# Autodesk Inventor assembly: LifterRight
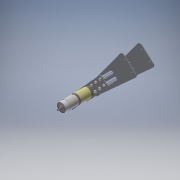
[picture p0: Inventor's stored thumbnail of the model, 180x180]
Saved by Autodesk Inventor 2017 (Build 210142000, 142)
## iProperties
Created: 2017-02-09
Part Number: LifterRight
Document SubType Name: Assembly
Designer: kingb
Author: kingb
## Documents named in this file (10)
- C:\Users\kingb\Desktop\CAD\LifterRight.iam
- C:\Users\kingb\Desktop\CAD\lifterMountMetal.ipt
- C:\Users\kingb\Desktop\CAD\newCoupler.ipt
- C:\Users\kingb\Desktop\CAD\Churro 3375.ipt
- C:\Users\kingb\Desktop\CAD\guidebar.ipt
- C:\Users\kingb\Desktop\CAD\10-32x0500_shcs_HX-SHCS 0.19-32x1.375x1-C.ipt
- C:\Users\kingb\Desktop\CAD\FHTS 0.25-20-0.75_FHTS 0.25-20-G-0.75-C.ipt
- C:\Users\kingb\Desktop\CAD\10-32 Nylock Nut.ipt
- C:\Users\kingb\Desktop\CAD\PG188withMotor.ipt
- C:\Users\kingb\Desktop\CAD\pG188Mount.ipt
## Components (30 placed, 9 different names)
1. lifterMountMetal:1 — Mate:5, Mate:6, Insert:12, Insert:14, Insert:15, Insert:16, Insert:17, Insert:26, Insert:27, Mate:11, Mate:12, Insert:30, Mate:18
2. newCoupler:1
3. Churro 3375:1 — Insert:31
4. Churro 3375:2 — Insert:34
5. Churro 3375:3 — Mate:5, Insert:33
6. Churro 3375:5 — Insert:32
7. guidebar:1 — Mate:6, Insert:24, Insert:25, Insert:28, Insert:29, Mate:11, Mate:12
8. Churro 3375:6 — Insert:36
9. Churro 3375:7 — Insert:35
10. 10-32x0500_shcs_HX-SHCS 0.19-32x1.375x1-C:1
11. 10-32x0500_shcs_HX-SHCS 0.19-32x1.375x1-C:2
12. FHTS 0.25-20-0.75_FHTS 0.25-20-G-0.75-C:1
13. FHTS 0.25-20-0.75_FHTS 0.25-20-G-0.75-C:2
14. FHTS 0.25-20-0.75_FHTS 0.25-20-G-0.75-C:3
15. FHTS 0.25-20-0.75_FHTS 0.25-20-G-0.75-C:4
16. FHTS 0.25-20-0.75_FHTS 0.25-20-G-0.75-C:5
17. FHTS 0.25-20-0.75_FHTS 0.25-20-G-0.75-C:6
18. FHTS 0.25-20-0.75_FHTS 0.25-20-G-0.75-C:7 — Insert:16
19. FHTS 0.25-20-0.75_FHTS 0.25-20-G-0.75-C:8 — Insert:17
20. FHTS 0.25-20-0.75_FHTS 0.25-20-G-0.75-C:9 — Insert:14
21. FHTS 0.25-20-0.75_FHTS 0.25-20-G-0.75-C:10 — Insert:15
22. FHTS 0.25-20-0.75_FHTS 0.25-20-G-0.75-C:11 — Insert:30
23. FHTS 0.25-20-0.75_FHTS 0.25-20-G-0.75-C:12 — Insert:12
24. 10-32x0500_shcs_HX-SHCS 0.19-32x1.375x1-C:3 — Insert:24
25. 10-32x0500_shcs_HX-SHCS 0.19-32x1.375x1-C:4 — Insert:25
26. 10-32 Nylock Nut:1 — Insert:27
27. 10-32 Nylock Nut:2 — Insert:26
28. lifterMountMetal:2 — Insert:28, Insert:29
29. PG188withMotor:1 — Angle:3, Mate:17, Mate:18
30. pG188Mount:1 — Angle:3, Mate:17, Insert:31, Insert:32, Insert:33, Insert:34, Insert:35, Insert:36
## Relationships (25: Insert 18, Mate 6, Angle 1)
- Mate:5: lifterMountMetal:1 ↔ Churro 3375:3
- Mate:6: lifterMountMetal:1 ↔ guidebar:1
- Insert:12: lifterMountMetal:1 ↔ FHTS 0.25-20-0.75_FHTS 0.25-20-G-0.75-C:12
- Insert:14: lifterMountMetal:1 ↔ FHTS 0.25-20-0.75_FHTS 0.25-20-G-0.75-C:9
- Insert:15: lifterMountMetal:1 ↔ FHTS 0.25-20-0.75_FHTS 0.25-20-G-0.75-C:10
- Insert:16: lifterMountMetal:1 ↔ FHTS 0.25-20-0.75_FHTS 0.25-20-G-0.75-C:7
- Insert:17: lifterMountMetal:1 ↔ FHTS 0.25-20-0.75_FHTS 0.25-20-G-0.75-C:8
- Insert:24: guidebar:1 ↔ 10-32x0500_shcs_HX-SHCS 0.19-32x1.375x1-C:3
- Insert:25: guidebar:1 ↔ 10-32x0500_shcs_HX-SHCS 0.19-32x1.375x1-C:4
- Insert:26: lifterMountMetal:1 ↔ 10-32 Nylock Nut:2
- Insert:27: lifterMountMetal:1 ↔ 10-32 Nylock Nut:1
- Insert:28: guidebar:1 ↔ lifterMountMetal:2
- Insert:29: guidebar:1 ↔ lifterMountMetal:2
- Mate:11 (-12.7 mm): lifterMountMetal:1 ↔ guidebar:1
- Mate:12: lifterMountMetal:1 ↔ guidebar:1
- Insert:30: lifterMountMetal:1 ↔ FHTS 0.25-20-0.75_FHTS 0.25-20-G-0.75-C:11
- Angle:3 (0 deg): PG188withMotor:1 ↔ pG188Mount:1
- Mate:17: PG188withMotor:1 ↔ pG188Mount:1
- Insert:31: Churro 3375:1 ↔ pG188Mount:1
- Insert:32: Churro 3375:5 ↔ pG188Mount:1
- Insert:33: Churro 3375:3 ↔ pG188Mount:1
- Insert:34: Churro 3375:2 ↔ pG188Mount:1
- Insert:35: Churro 3375:7 ↔ pG188Mount:1
- Insert:36: Churro 3375:6 ↔ pG188Mount:1
- Mate:18: lifterMountMetal:1 ↔ PG188withMotor:1
